# Autodesk Inventor assembly: Power bank
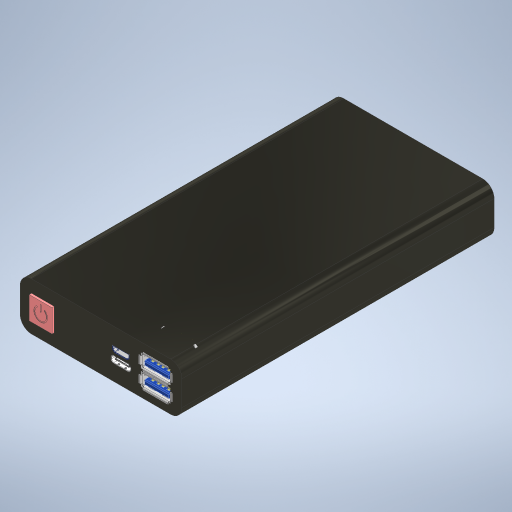
[picture p0: Inventor's stored thumbnail of the model, 512x512]
Saved by Autodesk Inventor 2023 (Build 270158000, 158)
## iProperties
Created: 2023-04-11
Part Number: Power bank
Document SubType Name: Assembly
Designer: ASARe-DAQ-PC
Author: ASARe-DAQ-PC
## Documents named in this file (5)
- D:\EB camera\model of EB camera\for manufacture\Power bank.iam
- D:\EB camera\model of EB camera\for manufacture\power bank.ipt
- D:\EB camera\model of EB camera\for manufacture\User Library-micro usb SMD.ipt
- D:\EB camera\model of EB camera\for manufacture\User Library-USB - C.ipt
- D:\EB camera\model of EB camera\for manufacture\User Library-USB-A-01.ipt
## Components (5 placed, 4 different names)
1. power bank:1 — Mate:1, Mate:2, Flush:1, Flush:2, Mate:3, Mate:4, Mate:5, Mate:6, Mate:7, Mate:8, Mate:9, Mate:10
2. User Library-micro usb SMD:1 — Mate:1, Mate:2, Flush:1
3. User Library-USB - C:1 — Flush:2, Mate:3, Mate:4
4. User Library-USB-A-01:1 — Mate:5, Mate:6, Mate:7
5. User Library-USB-A-01:2 — Mate:8, Mate:9, Mate:10
## Relationships (12: Mate 10, Flush 2)
- Mate:1: power bank:1 ↔ User Library-micro usb SMD:1
- Mate:2: power bank:1 ↔ User Library-micro usb SMD:1
- Flush:1: power bank:1 ↔ User Library-micro usb SMD:1
- Flush:2: power bank:1 ↔ User Library-USB - C:1
- Mate:3: power bank:1 ↔ User Library-USB - C:1
- Mate:4: power bank:1 ↔ User Library-USB - C:1
- Mate:5: power bank:1 ↔ User Library-USB-A-01:1
- Mate:6: power bank:1 ↔ User Library-USB-A-01:1
- Mate:7: power bank:1 ↔ User Library-USB-A-01:1
- Mate:8: power bank:1 ↔ User Library-USB-A-01:2
- Mate:9: power bank:1 ↔ User Library-USB-A-01:2
- Mate:10: power bank:1 ↔ User Library-USB-A-01:2
